# Autodesk Inventor assembly: Group
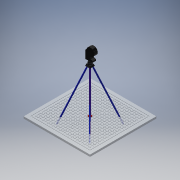
[picture p0: Inventor's stored thumbnail of the model, 180x180]
Saved by Autodesk Inventor 2018.2 (Build 222227000, 227)
## iProperties
Created: 2018-04-10
Part Number: Group
Material: Generisch
Document SubType Name: Assembly
Designer: Nick Koch
Author: Nick Koch
## Documents named in this file (5)
- C:\Users\Nick Koch\Desktop\Lehre\FHNW\Raytracing Modell\Group.iam
- C:\Users\Nick Koch\Desktop\Lehre\FHNW\Raytracing Modell\MiddleStick.ipt
- C:\Users\Nick Koch\Desktop\Lehre\FHNW\Raytracing Modell\Screen.ipt
- C:\Users\Nick Koch\Desktop\Lehre\FHNW\Raytracing Modell\Camera.ipt
- C:\Users\Nick Koch\Desktop\Lehre\FHNW\Raytracing Modell\blueStick.ipt
## Components (7 placed, 4 different names)
1. MiddleStick:1 — Passend:1, Passend:2, Passend:3, Passend:4, Passend:5, Passend:6, Passend:16
2. Screen:1 — Passend:1, Passend:2, Passend:3, Passend:16
3. Camera:1 — Passend:4, Passend:5, Passend:6, Passend:7, Passend:8, Passend:9, Passend:10, Passend:11, Passend:12, Passend:13, Passend:14, Passend:15, Passend:17, Passend:18, Passend:19
4. blueStick:1 — Passend:7, Passend:8, Passend:9
5. blueStick:2 — Passend:17, Passend:18, Passend:19
6. blueStick:3 — Passend:13, Passend:14, Passend:15
7. blueStick:4 — Passend:10, Passend:11, Passend:12
## Relationships (19: Mate 19)
- Passend:1 [Mate]: MiddleStick:1 ↔ Screen:1
- Passend:2 [Mate]: MiddleStick:1 ↔ Screen:1
- Passend:3 [Mate]: MiddleStick:1 ↔ Screen:1
- Passend:4 [Mate]: MiddleStick:1 ↔ Camera:1
- Passend:5 [Mate]: MiddleStick:1 ↔ Camera:1
- Passend:6 [Mate]: MiddleStick:1 ↔ Camera:1
- Passend:7 [Mate]: Camera:1 ↔ blueStick:1
- Passend:8 [Mate]: Camera:1 ↔ blueStick:1
- Passend:9 [Mate]: Camera:1 ↔ blueStick:1
- Passend:10 [Mate]: Camera:1 ↔ blueStick:4
- Passend:11 [Mate]: Camera:1 ↔ blueStick:4
- Passend:12 [Mate]: Camera:1 ↔ blueStick:4
- Passend:13 [Mate]: Camera:1 ↔ blueStick:3
- Passend:14 [Mate]: Camera:1 ↔ blueStick:3
- Passend:15 [Mate]: Camera:1 ↔ blueStick:3
- Passend:16 [Mate]: MiddleStick:1 ↔ Screen:1
- Passend:17 [Mate]: Camera:1 ↔ blueStick:2
- Passend:18 [Mate]: Camera:1 ↔ blueStick:2
- Passend:19 [Mate]: Camera:1 ↔ blueStick:2
